# Autodesk Inventor assembly: painel
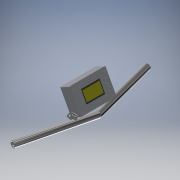
[picture p0: Inventor's stored thumbnail of the model, 180x180]
Saved by Autodesk Inventor 2019 (Build 230136000, 136)
## iProperties
Created: 2020-05-31
Part Number: painel
Document SubType Name: Assembly
Designer: luiza
Author: luiza
## Documents named in this file (10)
- G:\Meu Drive\Projetos\Projeto 2020 2021\Eletrônica 2020-2021\Projeção mecânica\Painel\painel.iam
- G:\Meu Drive\Projetos\Projeto 2020 2021\Eletrônica 2020-2021\Projeção mecânica\Painel\Caixa Painel.ipt
- G:\Meu Drive\Projetos\Projeto 2020 2021\Eletrônica 2020-2021\Projeção mecânica\Painel\Espaçadores.ipt
- G:\Meu Drive\Projetos\Projeto 2020 2021\Eletrônica 2020-2021\Projeção mecânica\Painel\Fixação Painel.ipt
- G:\Meu Drive\Projetos\Projeto 2020 2021\Eletrônica 2020-2021\Projeção mecânica\Painel\Tampa Painel.ipt
- G:\Meu Drive\Projetos\Projeto 2020 2021\Eletrônica 2020-2021\Projeção mecânica\Painel\LCD12864_st7920.iam
- G:\Meu Drive\Projetos\Projeto 2020 2021\Suspensão & Direção 2020_2021\Geometrias\Geometria Suspensão e Direção.iam
- G:\Meu Drive\Projetos\Projeto 2020 2021\Eletrônica 2020-2021\Projeção mecânica\Painel\painel\Frame\Frame0001.iam
- G:\Meu Drive\Projetos\Projeto 2020 2021\Eletrônica 2020-2021\Projeção mecânica\Painel\AMP 3 position.ipt
- G:\Meu Drive\Projetos\Projeto 2020 2021\Eletrônica 2020-2021\Projeção mecânica\Caixas\Módulo Central\AMP 3 position.ipt
## Components (15 placed, 8 different names)
1. Tampa Painel:1 — Mate:4, Flush:3, Mate:13, Mate:14, Mate:19, Mate:20
2. LCD12864_st7920:1 [sub-assembly] — Flush:3, Mate:5, Mate:6, Mate:7, Mate:8, Mate:13, Mate:14, Mate:15, Mate:16, Mate:17, Mate:18
3. Caixa Painel:1 — Mate:2, Mate:3, Angle:1, Mate:4, Mate:19, Mate:20, Flush:22, Mate:22, Mate:23, Mate:24, Mate:25, Mate:26, Mate:28, Mate:29, Mate:31, Mate:32, Mate:33, Mate:34, Mate:35
4. Espaçadores:1 — Mate:6, Mate:17
5. Espaçadores:2 — Mate:5, Mate:16
6. Espaçadores:3 — Mate:8, Mate:18
7. Espaçadores:4 — Mate:7, Mate:15
8. Geometria Suspensão e Direção:1 [sub-assembly]
9. Fixação Painel:1 — Mate:1, Flush:1, Flush:2
10. Fixação Painel:2 — Mate:1, Flush:1, Flush:2, Mate:2, Mate:3, Angle:1, Mate:21
11. Frame0001:1 [sub-assembly] — Flush:22, Mate:21
12. AMP 3 position:1 — Mate:22, Mate:23, Mate:24
13. AMP 3 position:2 — Mate:25, Mate:26, Mate:35
14. AMP 3 position:3 — Mate:28, Mate:29, Mate:34
15. AMP 3 position:4 — Mate:31, Mate:32, Mate:33
## Relationships (34: Mate 29, Flush 4, Angle 1)
- Mate:1 (150 mm): Fixação Painel:1 ↔ Fixação Painel:2
- Flush:1: Fixação Painel:1 ↔ Fixação Painel:2
- Flush:2: Fixação Painel:1 ↔ Fixação Painel:2
- Mate:2: Caixa Painel:1 ↔ Fixação Painel:2
- Mate:3: Caixa Painel:1 ↔ Fixação Painel:2
- Angle:1 (-90 deg): Caixa Painel:1 ↔ Fixação Painel:2
- Mate:4: Tampa Painel:1 ↔ Caixa Painel:1
- Flush:3: Tampa Painel:1 ↔ LCD12864_st7920:1
- Mate:5: LCD12864_st7920:1 ↔ Espaçadores:2
- Mate:6: LCD12864_st7920:1 ↔ Espaçadores:1
- Mate:7: LCD12864_st7920:1 ↔ Espaçadores:4
- Mate:8: LCD12864_st7920:1 ↔ Espaçadores:3
- Mate:13 (0.2 mm): Tampa Painel:1 ↔ LCD12864_st7920:1
- Mate:14 (0.2 mm): Tampa Painel:1 ↔ LCD12864_st7920:1
- Mate:15: LCD12864_st7920:1 ↔ Espaçadores:4
- Mate:16: LCD12864_st7920:1 ↔ Espaçadores:2
- Mate:17: LCD12864_st7920:1 ↔ Espaçadores:1
- Mate:18: LCD12864_st7920:1 ↔ Espaçadores:3
- Mate:19 (1 mm): Tampa Painel:1 ↔ Caixa Painel:1
- Mate:20 (1 mm): Tampa Painel:1 ↔ Caixa Painel:1
- Flush:22 (75 mm): Caixa Painel:1 ↔ Frame0001:1
- Mate:21: Fixação Painel:2 ↔ Frame0001:1
- Mate:22: Caixa Painel:1 ↔ AMP 3 position:1
- Mate:23: Caixa Painel:1 ↔ AMP 3 position:1
- Mate:24 (0.1 mm): Caixa Painel:1 ↔ AMP 3 position:1
- Mate:25: Caixa Painel:1 ↔ AMP 3 position:2
- Mate:26 (0.1 mm): Caixa Painel:1 ↔ AMP 3 position:2
- Mate:28: Caixa Painel:1 ↔ AMP 3 position:3
- Mate:29 (0.1 mm): Caixa Painel:1 ↔ AMP 3 position:3
- Mate:31: Caixa Painel:1 ↔ AMP 3 position:4
- Mate:32 (0.1 mm): Caixa Painel:1 ↔ AMP 3 position:4
- Mate:33: Caixa Painel:1 ↔ AMP 3 position:4
- Mate:34: Caixa Painel:1 ↔ AMP 3 position:3
- Mate:35: Caixa Painel:1 ↔ AMP 3 position:2
